# Autodesk Inventor assembly: Robot-ver2-1111-2020
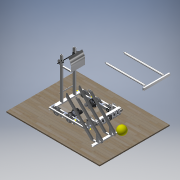
[picture p0: Inventor's stored thumbnail of the model, 180x180]
Saved by Autodesk Inventor 2018 (Build 220112000, 112)
## iProperties
Created: 2020-01-25
Part Number: Robot-ver2-1111-2020
Document SubType Name: Assembly
Designer: JMHal
Author: JMHal
## Documents named in this file (6)
- E:\GrabCAD\Power Hawks CAD\2020 Infinite Recharge\Final Robot Assembly\Robot-ver2-1111-2020.iam
- E:\GrabCAD\Power Hawks CAD\2020 Infinite Recharge\Chassis\Assembly\Chassis-ver13-1111-2019.iam
- E:\GrabCAD\Power Hawks CAD\2020 Infinite Recharge\Intake\Assemblies\IntakeAssembly-ver1-1111-2020.iam
- E:\GrabCAD\Power Hawks CAD\2020 Infinite Recharge\Lift\Assemblies\PistonLift-ver1-1111-2020.iam
- E:\GrabCAD\Power Hawks CAD\2020 Infinite Recharge\Shooting\Assemblies\ShooterPrototype-ver2-1111-2019.iam
- E:\GrabCAD\Power Hawks CAD\2020 Infinite Recharge\Storage\Assemblies\StorageAssembly.ver4-1111-2020.iam
## Components (5 placed, 5 different names)
1. Chassis-ver13-1111-2019:1 [sub-assembly] — Mate:1, Mate:2, Mate:3, Flush:1, Mate:4, Flush:2, Mate:5, Angle:1
2. IntakeAssembly-ver1-1111-2020:1 [sub-assembly] — Mate:3, Flush:1
3. PistonLift-ver1-1111-2020:1 [sub-assembly]
4. ShooterPrototype-ver2-1111-2019:1 [sub-assembly] — Mate:4, Flush:2
5. StorageAssembly.ver4-1111-2020:1 [sub-assembly] — Mate:5, Angle:1
## Relationships (8: Mate 5, Flush 2, Angle 1)
- Mate:1: Chassis-ver13-1111-2019:1
- Mate:2: Chassis-ver13-1111-2019:1
- Mate:3: Chassis-ver13-1111-2019:1 ↔ IntakeAssembly-ver1-1111-2020:1
- Flush:1: Chassis-ver13-1111-2019:1 ↔ IntakeAssembly-ver1-1111-2020:1
- Mate:4: Chassis-ver13-1111-2019:1 ↔ ShooterPrototype-ver2-1111-2019:1
- Flush:2: Chassis-ver13-1111-2019:1 ↔ ShooterPrototype-ver2-1111-2019:1
- Mate:5: Chassis-ver13-1111-2019:1 ↔ StorageAssembly.ver4-1111-2020:1
- Angle:1 (0 deg): Chassis-ver13-1111-2019:1 ↔ StorageAssembly.ver4-1111-2020:1
